# Autodesk Inventor assembly: engine 101 standing model (no movement)
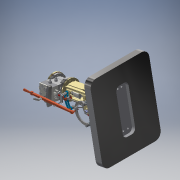
[picture p0: Inventor's stored thumbnail of the model, 180x180]
Saved by Autodesk Inventor 2017 (Build 210142000, 142)
## iProperties
Created: 2018-11-11
Part Number: engine 101 standing model (no movement)
Document SubType Name: Assembly
Designer: User
Author: User
## Documents named in this file (53)
- E:\Sahil's engine\engine 101 standing model (no movement).iam
- E:\Sahil's engine\reverse gear fly wheel.ipt
- E:\Sahil's engine\reverse gear crankshaft outer rod.ipt
- E:\Sahil's engine\reverse gear crankshaft counter weight 2.ipt
- E:\Sahil's engine\reverse gear bearing keeper.ipt
- E:\Sahil's engine\reverse gear connecting rod 1.ipt
- E:\Sahil's engine\reverse gear crankshaft center rod.ipt
- E:\Sahil's engine\reverse gear crank rod 1.ipt
- E:\Sahil's engine\reverse gear crankrod pin 1.ipt
- E:\Sahil's engine\reverse gear cross head 1.ipt
- E:\Sahil's engine\reverse gear pistion rod.ipt
- E:\Sahil's engine\reverse gear piston.ipt
- E:\Sahil's engine\reverse gear  upper base bearing holder 1.ipt
- E:\Sahil's engine\reverse gear lower base bearing holder.ipt
- E:\Sahil's engine\reverse gear lower cylinder ream 1.ipt
- E:\Sahil's engine\reverse gear eccentric 1.ipt
- E:\Sahil's engine\reverse gear base cast 2.ipt
- E:\Sahil's engine\reverse gear stand.ipt
- E:\Sahil's engine\reverse gear lower cylinder cover.ipt
- E:\Sahil's engine\reverse gear cylinder.ipt
- E:\Sahil's engine\reverse gear steam chest.ipt
- E:\Sahil's engine\reverse gear steam chest cover.ipt
- E:\Sahil's engine\reverse gear gear link.ipt
- E:\Sahil's engine\reverse gear link stud.ipt
- C:\Users\User\Documents\engine\Good copy engine Sahil\reverse gear link lever.ipt
- E:\Sahil's engine\reverse gear standard 101.ipt
- E:\Sahil's engine\reverse gear blands.ipt
- C:\Users\User\Documents\engine\Good copy engine Sahil\reverse gear steam chest rod valve.ipt
- E:\Sahil's engine\reverse gear reverse gear.ipt
- E:\Sahil's engine\reverse gear link block.ipt
- E:\Sahil's engine\reverse gear essentric rod 2.ipt
- E:\Sahil's engine\reverse gear trap holders.ipt
- E:\Sahil's engine\reverse gear lower trap.ipt
- E:\Sahil's engine\reverse gear drag link.ipt
- E:\Sahil's engine\reverse gear link rod.ipt
- E:\Sahil's engine\reverse gear lever ring stud.ipt
- E:\Sahil's engine\reverse gear reverse lever ring.ipt
- E:\Sahil's engine\reverse gear cylinder piping connector 2.ipt
- E:\Sahil's engine\reverse gear rever lever.ipt
- C:\Users\User\Documents\Inventor\Content Center Files\R2017\en-US\DIN 84\DIN 84 - M3 x 4.ipt
- C:\Users\User\Documents\Inventor\Content Center Files\R2017\en-US\DIN 84\DIN 84 - M4 x 14.ipt
- C:\Users\User\Documents\Inventor\Content Center Files\R2017\en-US\CNS 4472\CNS 4472 - M 6 x 1.ipt
- C:\Users\User\Documents\Inventor\Content Center Files\R2017\en-US\AS 1421(1)\AS 1421 - M3x5 Cone Point.ipt
- C:\Users\User\Documents\Inventor\Content Center Files\R2017\en-US\AS 1427(03)\AS 1427 - M2.5 x 5(1).ipt
- C:\Users\User\Documents\Inventor\Content Center Files\R2017\en-US\CSN 02 1174  A\CSN 02 1174 - A M3 x 20.ipt
- C:\Users\User\Documents\Inventor\Content Center Files\R2017\en-US\CSN 02 1174  A\CSN 02 1174 - A M3 x 14.ipt
- E:\Sahil's engine\reverse gear up cylinder packing.ipt
- C:\Users\User\Documents\Inventor\Content Center Files\R2017\en-US\AS 1427(03)\AS 1427 - M2 x 10(1).ipt
- E:\Sahil's engine\reverse gear upper cover.ipt
- C:\Users\User\Documents\Inventor\Content Center Files\R2017\en-US\AS 1427(03)\AS 1427 - M2 x 8(1).ipt
- C:\Users\User\Documents\Inventor\Content Center Files\R2017\en-US\AS 1427(03)\AS 1427 - M2 x 6(1).ipt
- C:\Users\User\Documents\Inventor\Content Center Files\R2017\en-US\AS 1427(03)\AS 1427 - M3.5 x 6(1).ipt
- C:\Users\User\Documents\Inventor\Content Center Files\R2017\en-US\AS 1427(03)\AS 1427 - M2 x 20(1).ipt
## Components (109 placed, 52 different names)
1. reverse gear crankshaft outer rod:1 — Insert:2, Insert:21, Rotation:2, Rotation:3
2. reverse gear crankshaft counter weight 2:1 — Insert:2, Rotation:1, Insert:86
3. reverse gear connecting rod 1:2 — Mate:1, Flush:1, Flush:2, Mate:2, Flush:3, Flush:4
4. reverse gear connecting rod 1:3 — Mate:1, Flush:1, Flush:2, Mate:3, Flush:5, Flush:6
5. reverse gear bearing keeper:2 — Mate:2, Flush:3, Flush:4
6. reverse gear crankshaft counter weight 2:2 — Insert:6, Insert:84, Insert:85
7. reverse gear crankshaft outer rod:2 — Insert:6, Insert:12, Insert:14, Insert:15
8. reverse gear crank rod 1:1 — Mate:3, Flush:5, Flush:6, Insert:7, Insert:8, Insert:82, Insert:83
9. reverse gear crankrod pin 1:1 — Insert:7
10. reverse gear cross head 1:1 — Insert:8, Insert:9
11. reverse gear pistion rod:1 — Insert:9, Insert:10, Insert:13
12. reverse gear piston:1 — Insert:10, Insert:30
13. reverse gear  upper base bearing holder 1:1 — Mate:4, Flush:7, Flush:8, Flush:26, Insert:68, Insert:78, Insert:79, Insert:80, Insert:81
14. reverse gear  upper base bearing holder 1:2 — Mate:5, Flush:9, Flush:10, Insert:12, Flush:12, Flush:13, Insert:69, Insert:74, Insert:75, Insert:76, Insert:77, Rotation/Translation:6, Rotation/Translation:7, Rotation/Translation:8, Rotation/Translation:9, Rotation/Translation:10, Rotation/Translation:11, Rotation/Translation:13
15. reverse gear lower base bearing holder:1 — Mate:4, Flush:7, Flush:8, Mate:6, Flush:25, Rotation:1
16. reverse gear lower base bearing holder:2 — Mate:5, Flush:9, Flush:10, Mate:7, Flush:11
17. reverse gear lower cylinder ream 1:1 — Insert:13, Insert:16
18. reverse gear eccentric 1:1 — Insert:14, Insert:31
19. reverse gear eccentric 1:2 — Insert:15, Insert:33
20. reverse gear base cast 2:1 — Mate:6, Mate:7, Flush:11, Flush:12, Flush:13, Mate:8, Flush:14, Flush:15, Flush:20, Flush:21, Flush:22, Flush:25, Flush:26, Insert:41, Insert:43, Rotation:9, Insert:56, Insert:57, Insert:58, Insert:59, Rotation/Translation:14
21. reverse gear stand:1 — Mate:8, Flush:14, Flush:15
22. reverse gear lower cylinder cover:1 — Insert:16
23. reverse gear steam chest:1 — Mate:10, Flush:18, Flush:19, Insert:23, Mate:19, Flush:28, Flush:29, Insert:46
24. reverse gear steam chest cover:1 — Mate:10, Flush:18, Flush:19, Mate:11, Mate:12, Mate:14, Mate:15, Insert:102, Insert:103, Insert:104, Insert:105, Insert:106, Insert:107
25. reverse gear gear link:1 — Mate:11, Mate:12, Mate:14, Mate:15, Rotation:4, Insert:100, Insert:101
26. reverse gear link lever:1 — Rotation:5, Insert:111
27. reverse gear standard 101:1 — Flush:20, Flush:21, Flush:22, Rotation:6, Rotation:7, Insert:50, Insert:51, Insert:52, Insert:53, Insert:54, Insert:55, Rotation:12, Rotation/Translation:1, Rotation/Translation:2, Rotation/Translation:3, Rotation/Translation:4, Rotation/Translation:5, Rotation:15
28. reverse gear fly wheel:1 — Insert:21, Rotation:2, Rotation:3
29. reverse gear blands:1 — Insert:23, Insert:35
30. reverse gear steam chest rod valve:1 — Mate:16, Mate:17, Insert:25, Insert:35
31. reverse gear reverse gear:1 — Insert:26, Insert:28, Rotation:8, Insert:37
32. reverse gear link stud:2 — Insert:25
33. reverse gear link block:1 — Mate:16, Mate:17
34. reverse gear link stud:3 — Insert:26, Insert:36
35. reverse gear link stud:4 — Insert:28, Rotation:8
36. reverse gear cylinder:1 — Insert:30, Mate:19, Flush:28, Flush:29, Rotation:4, Rotation:5, Rotation:6, Rotation:7, Insert:45, Mate:22, Insert:95, Insert:96, Insert:97, Insert:98, Insert:99, Rotation:15
37. reverse gear trap holders:1 — Insert:31, Mate:20, Flush:30, Insert:32, Insert:70, Insert:72
38. reverse gear lower trap:1 — Mate:20, Flush:30
39. reverse gear essentric rod 2:2 — Insert:32, Insert:36
40. reverse gear trap holders:2 — Insert:33, Mate:21, Flush:31, Insert:34, Insert:71, Insert:73
41. reverse gear lower trap:2 — Mate:21, Flush:31
42. reverse gear essentric rod 2:3 — Insert:34
43. reverse gear drag link:1 — Insert:38
44. reverse gear link rod:1 — Insert:37, Insert:38
45. reverse gear reverse lever ring:1 — Insert:42, Rotation:9, Insert:44
46. reverse gear lever ring stud:1 — Insert:41, Insert:42
47. reverse gear lever ring stud:2 — Insert:43
48. reverse gear link stud:6 — Insert:44, Insert:108
49. reverse gear cylinder piping connector 2:1 — Insert:45
50. reverse gear cylinder piping connector 2:2 — Insert:46
51. DIN 84 - replaced by DIN EN ISO 1207 M3 x 4:1 — Insert:50, Rotation:12, Rotation/Translation:1
52. DIN 84 - replaced by DIN EN ISO 1207 M3 x 4:2 — Insert:55, Rotation/Translation:4
53. DIN 84 - replaced by DIN EN ISO 1207 M3 x 4:3 — Insert:54, Rotation/Translation:5
54. DIN 84 - replaced by DIN EN ISO 1207 M3 x 4:4 — Insert:51, Rotation/Translation:2
55. DIN 84 - replaced by DIN EN ISO 1207 M3 x 4:5 — Insert:53
56. DIN 84 - replaced by DIN EN ISO 1207 M3 x 4:6 — Insert:52, Rotation/Translation:3
57. DIN 84 - replaced by DIN EN ISO 1207 M4 x 14:1 — Insert:58, Insert:60
58. DIN 84 - replaced by DIN EN ISO 1207 M4 x 14:2 — Insert:59, Insert:61
59. DIN 84 - replaced by DIN EN ISO 1207 M4 x 14:3 — Insert:56, Insert:62
60. DIN 84 - replaced by DIN EN ISO 1207 M4 x 14:4 — Insert:57, Insert:63
61. CNS 4472 M 6:1 — Insert:60
62. CNS 4472 M 6:2 — Insert:61
63. CNS 4472 M 6:3 — Insert:62
64. CNS 4472 M 6:4 — Insert:63
65. DIN 84 - replaced by DIN EN ISO 1207 M3 x 4:7 — Insert:68
66. DIN 84 - replaced by DIN EN ISO 1207 M3 x 4:8 — Insert:69
67. AS 1421 Cone Point - Metric M3x5 Cone Point:1 — Insert:73
68. AS 1421 Cone Point - Metric M3x5 Cone Point:2 — Insert:71
69. AS 1421 Cone Point - Metric M3x5 Cone Point:3 — Insert:72
70. AS 1421 Cone Point - Metric M3x5 Cone Point:4 — Insert:70
71. AS 1427 - Metric M2.5 x 5:1 — Insert:74, Rotation:14, Rotation/Translation:11, Rotation/Translation:12
72. AS 1427 - Metric M2.5 x 5:2 — Insert:75, Rotation:14, Rotation/Translation:12, Rotation/Translation:13
73. AS 1427 - Metric M2.5 x 5:3 — Insert:76, Rotation/Translation:6, Rotation/Translation:7, Rotation:13
74. AS 1427 - Metric M2.5 x 5:4 — Insert:77, Rotation:13, Rotation/Translation:8, Rotation/Translation:9, Rotation/Translation:10
75. AS 1427 - Metric M2.5 x 5:5 — Insert:78
76. AS 1427 - Metric M2.5 x 5:6 — Insert:80
77. AS 1427 - Metric M2.5 x 5:7 — Insert:79
78. AS 1427 - Metric M2.5 x 5:8 — Insert:81
79. CSN 02 1174 A A M3 x 20:1 — Insert:83
80. CSN 02 1174 A A M3 x 20:2 — Insert:82
81. reverse gear crankshaft center rod:2 — Insert:84
82. CSN 02 1174 A A M3 x 14:1 — Insert:86
83. CSN 02 1174 A A M3 x 14:2 — Insert:85
84. reverse gear up cylinder packing:1 — Mate:22, Mate:23
85. reverse gear upper cover:1 — Mate:23, Insert:87, Insert:88, Insert:89, Insert:90, Insert:91, Insert:92, Insert:93, Insert:94
86. AS 1427 - Metric M2 x 8:1 — Insert:93
87. AS 1427 - Metric M2 x 8:2 — Insert:90
88. AS 1427 - Metric M2 x 8:3 — Insert:88
89. AS 1427 - Metric M2 x 8:4 — Insert:87
90. AS 1427 - Metric M2 x 8:6 — Insert:91
91. AS 1427 - Metric M2 x 8:7 — Insert:92
92. AS 1427 - Metric M2 x 8:8 — Insert:89
93. AS 1427 - Metric M2 x 10:1 — Insert:94
94. AS 1427 - Metric M2 x 6:2 — Insert:97
95. AS 1427 - Metric M2 x 6:4 — Insert:95
96. AS 1427 - Metric M2 x 6:6 — Insert:99
97. AS 1427 - Metric M2 x 6:7 — Insert:98
98. AS 1427 - Metric M2 x 6:8 — Insert:96
99. AS 1427 - Metric M3.5 x 6:1 — Insert:102
100. AS 1427 - Metric M3.5 x 6:2 — Insert:101
101. AS 1427 - Metric M3.5 x 6:3 — Insert:104
102. AS 1427 - Metric M3.5 x 6:4 — Insert:100
103. AS 1427 - Metric M3.5 x 6:5 — Insert:105
104. AS 1427 - Metric M3.5 x 6:6 — Insert:103
105. AS 1427 - Metric M3.5 x 6:7 — Insert:107
106. AS 1427 - Metric M3.5 x 6:8 — Insert:106
107. reverse gear rever lever:1 — Insert:108, Insert:109, Insert:110, Rotation/Translation:14
108. AS 1427 - Metric M2 x 20:1 — Insert:110, Insert:111
109. AS 1427 - Metric M2 x 20:2 — Insert:109
## Relationships (162: Insert 89, Flush 26, Mate 20, RelateRotateTranslate 14, RelateRotation 13)
- Insert:2 (-7 mm): reverse gear crankshaft outer rod:1 ↔ reverse gear crankshaft counter weight 2:1
- Mate:1: reverse gear connecting rod 1:2 ↔ reverse gear connecting rod 1:3
- Flush:1: reverse gear connecting rod 1:2 ↔ reverse gear connecting rod 1:3
- Flush:2: reverse gear connecting rod 1:2 ↔ reverse gear connecting rod 1:3
- Mate:2: reverse gear connecting rod 1:2 ↔ reverse gear bearing keeper:2
- Flush:3: reverse gear connecting rod 1:2 ↔ reverse gear bearing keeper:2
- Flush:4: reverse gear connecting rod 1:2 ↔ reverse gear bearing keeper:2
- Insert:6: reverse gear crankshaft counter weight 2:2 ↔ reverse gear crankshaft outer rod:2
- Mate:3: reverse gear connecting rod 1:3 ↔ reverse gear crank rod 1:1
- Flush:5: reverse gear connecting rod 1:3 ↔ reverse gear crank rod 1:1
- Flush:6: reverse gear connecting rod 1:3 ↔ reverse gear crank rod 1:1
- Insert:7 (-20 mm): reverse gear crank rod 1:1 ↔ reverse gear crankrod pin 1:1
- Insert:8: reverse gear crank rod 1:1 ↔ reverse gear cross head 1:1
- Insert:9 (-7.5 mm): reverse gear cross head 1:1 ↔ reverse gear pistion rod:1
- Insert:10 (7 mm): reverse gear pistion rod:1 ↔ reverse gear piston:1
- Mate:4: reverse gear  upper base bearing holder 1:1 ↔ reverse gear lower base bearing holder:1
- Flush:7 (7 mm): reverse gear  upper base bearing holder 1:1 ↔ reverse gear lower base bearing holder:1
- Flush:8: reverse gear  upper base bearing holder 1:1 ↔ reverse gear lower base bearing holder:1
- Mate:5: reverse gear  upper base bearing holder 1:2 ↔ reverse gear lower base bearing holder:2
- Flush:9 (7 mm): reverse gear  upper base bearing holder 1:2 ↔ reverse gear lower base bearing holder:2
- Flush:10: reverse gear  upper base bearing holder 1:2 ↔ reverse gear lower base bearing holder:2
- Insert:12 (27 mm): reverse gear crankshaft outer rod:2 ↔ reverse gear  upper base bearing holder 1:2
- Insert:13 (-5 mm): reverse gear pistion rod:1 ↔ reverse gear lower cylinder ream 1:1
- Insert:14 (13 mm): reverse gear crankshaft outer rod:2 ↔ reverse gear eccentric 1:1
- Insert:15 (5 mm): reverse gear crankshaft outer rod:2 ↔ reverse gear eccentric 1:2
- Mate:6: reverse gear lower base bearing holder:1 ↔ reverse gear base cast 2:1
- Mate:7: reverse gear lower base bearing holder:2 ↔ reverse gear base cast 2:1
- Flush:11: reverse gear lower base bearing holder:2 ↔ reverse gear base cast 2:1
- Flush:12: reverse gear  upper base bearing holder 1:2 ↔ reverse gear base cast 2:1
- Flush:13 (29 mm): reverse gear  upper base bearing holder 1:2 ↔ reverse gear base cast 2:1
- Mate:8: reverse gear base cast 2:1 ↔ reverse gear stand:1
- Flush:14 (55 mm): reverse gear base cast 2:1 ↔ reverse gear stand:1
- Flush:15 (59 mm): reverse gear base cast 2:1 ↔ reverse gear stand:1
- Insert:16 (1 mm): reverse gear lower cylinder ream 1:1 ↔ reverse gear lower cylinder cover:1
- Mate:10: reverse gear steam chest:1 ↔ reverse gear steam chest cover:1
- Flush:18: reverse gear steam chest:1 ↔ reverse gear steam chest cover:1
- Flush:19: reverse gear steam chest:1 ↔ reverse gear steam chest cover:1
- Mate:11: reverse gear steam chest cover:1 ↔ reverse gear gear link:1
- Mate:12: reverse gear steam chest cover:1 ↔ reverse gear gear link:1
- Flush:20 (12 mm): reverse gear base cast 2:1 ↔ reverse gear standard 101:1
- Flush:21 (0.5 mm): reverse gear base cast 2:1 ↔ reverse gear standard 101:1
- Flush:22 (-3.9 mm): reverse gear base cast 2:1 ↔ reverse gear standard 101:1
- Mate:14: reverse gear steam chest cover:1 ↔ reverse gear gear link:1
- Mate:15: reverse gear steam chest cover:1 ↔ reverse gear gear link:1
- Flush:25: reverse gear lower base bearing holder:1 ↔ reverse gear base cast 2:1
- Flush:26 (29 mm): reverse gear  upper base bearing holder 1:1 ↔ reverse gear base cast 2:1
- Rotation:1 [RelateRotation] (1 ul): reverse gear crankshaft counter weight 2:1 ↔ reverse gear lower base bearing holder:1
- Insert:21 (-8 mm): reverse gear crankshaft outer rod:1 ↔ reverse gear fly wheel:1
- Rotation:2 [RelateRotation] (10.25 ul): reverse gear crankshaft outer rod:1 ↔ reverse gear fly wheel:1
- Rotation:3 [RelateRotation] (10.25 ul): reverse gear crankshaft outer rod:1 ↔ reverse gear fly wheel:1
- Insert:23 (-8 mm): reverse gear steam chest:1 ↔ reverse gear blands:1
- Mate:16: reverse gear steam chest rod valve:1 ↔ reverse gear link block:1
- Mate:17: reverse gear steam chest rod valve:1 ↔ reverse gear link block:1
- Insert:25 (-13 mm): reverse gear steam chest rod valve:1 ↔ reverse gear link stud:2
- Insert:26 (-10 mm): reverse gear reverse gear:1 ↔ reverse gear link stud:3
- Insert:28 (-10 mm): reverse gear reverse gear:1 ↔ reverse gear link stud:4
- Insert:30 (-23 mm): reverse gear piston:1 ↔ reverse gear cylinder:1
- Mate:19: reverse gear steam chest:1 ↔ reverse gear cylinder:1
- Flush:28: reverse gear steam chest:1 ↔ reverse gear cylinder:1
- Flush:29: reverse gear steam chest:1 ↔ reverse gear cylinder:1
- Rotation:4 [RelateRotation] (1 ul): reverse gear gear link:1 ↔ reverse gear cylinder:1
- Rotation:5 [RelateRotation] (1 ul): reverse gear link lever:1 ↔ reverse gear cylinder:1
- Rotation:6 [RelateRotation] (1 ul): reverse gear standard 101:1 ↔ reverse gear cylinder:1
- Rotation:7 [RelateRotation] (1 ul): reverse gear standard 101:1 ↔ reverse gear cylinder:1
- Insert:31 (-1.6 mm): reverse gear eccentric 1:1 ↔ reverse gear trap holders:1
- Mate:20: reverse gear trap holders:1 ↔ reverse gear lower trap:1
- Flush:30: reverse gear trap holders:1 ↔ reverse gear lower trap:1
- Insert:32 (-3 mm): reverse gear trap holders:1 ↔ reverse gear essentric rod 2:2
- Insert:33: reverse gear eccentric 1:2 ↔ reverse gear trap holders:2
- Mate:21: reverse gear trap holders:2 ↔ reverse gear lower trap:2
- Flush:31: reverse gear trap holders:2 ↔ reverse gear lower trap:2
- Insert:34 (-3 mm): reverse gear trap holders:2 ↔ reverse gear essentric rod 2:3
- Insert:35 (-40 mm): reverse gear blands:1 ↔ reverse gear steam chest rod valve:1
- Insert:36 (-6 mm): reverse gear link stud:3 ↔ reverse gear essentric rod 2:2
- Rotation:8 [RelateRotation] (1 ul): reverse gear reverse gear:1 ↔ reverse gear link stud:4
- Insert:37 (4.5 mm): reverse gear reverse gear:1 ↔ reverse gear link rod:1
- Insert:38 (-4 mm): reverse gear drag link:1 ↔ reverse gear link rod:1
- Insert:41: reverse gear base cast 2:1 ↔ reverse gear lever ring stud:1
- Insert:42: reverse gear reverse lever ring:1 ↔ reverse gear lever ring stud:1
- Insert:43: reverse gear base cast 2:1 ↔ reverse gear lever ring stud:2
- Rotation:9 [RelateRotation] (1 ul): reverse gear base cast 2:1 ↔ reverse gear reverse lever ring:1
- Insert:44 (-8 mm): reverse gear reverse lever ring:1 ↔ reverse gear link stud:6
- Insert:45: reverse gear cylinder:1 ↔ reverse gear cylinder piping connector 2:1
- Insert:46 (9 mm): reverse gear steam chest:1 ↔ reverse gear cylinder piping connector 2:2
- Insert:50 (-3.6 mm): reverse gear standard 101:1 ↔ DIN 84 - replaced by DIN EN ISO 1207 M3 x 4:1
- Insert:51 (-3.6 mm): reverse gear standard 101:1 ↔ DIN 84 - replaced by DIN EN ISO 1207 M3 x 4:4
- Insert:52 (-3.6 mm): reverse gear standard 101:1 ↔ DIN 84 - replaced by DIN EN ISO 1207 M3 x 4:6
- Insert:53 (-3.6 mm): reverse gear standard 101:1 ↔ DIN 84 - replaced by DIN EN ISO 1207 M3 x 4:5
- Insert:54 (-3.6 mm): reverse gear standard 101:1 ↔ DIN 84 - replaced by DIN EN ISO 1207 M3 x 4:3
- Insert:55 (-3.6 mm): reverse gear standard 101:1 ↔ DIN 84 - replaced by DIN EN ISO 1207 M3 x 4:2
- Rotation:12 [RelateRotation] (1 ul): reverse gear standard 101:1 ↔ DIN 84 - replaced by DIN EN ISO 1207 M3 x 4:1
- Rotation/Translation:1 [RelateRotateTranslate] (1 mm): reverse gear standard 101:1 ↔ DIN 84 - replaced by DIN EN ISO 1207 M3 x 4:1
- Rotation/Translation:2 [RelateRotateTranslate] (1 mm): reverse gear standard 101:1 ↔ DIN 84 - replaced by DIN EN ISO 1207 M3 x 4:4
- Rotation/Translation:3 [RelateRotateTranslate] (1 mm): reverse gear standard 101:1 ↔ DIN 84 - replaced by DIN EN ISO 1207 M3 x 4:6
- Rotation/Translation:4 [RelateRotateTranslate] (1 mm): reverse gear standard 101:1 ↔ DIN 84 - replaced by DIN EN ISO 1207 M3 x 4:2
- Rotation/Translation:5 [RelateRotateTranslate] (1 mm): reverse gear standard 101:1 ↔ DIN 84 - replaced by DIN EN ISO 1207 M3 x 4:3
- Insert:56 (-12.4 mm): reverse gear base cast 2:1 ↔ DIN 84 - replaced by DIN EN ISO 1207 M4 x 14:3
- Insert:57 (-12.4 mm): reverse gear base cast 2:1 ↔ DIN 84 - replaced by DIN EN ISO 1207 M4 x 14:4
- Insert:58 (-12.8 mm): reverse gear base cast 2:1 ↔ DIN 84 - replaced by DIN EN ISO 1207 M4 x 14:1
- Insert:59 (-12.8 mm): reverse gear base cast 2:1 ↔ DIN 84 - replaced by DIN EN ISO 1207 M4 x 14:2
- Insert:60 (4 mm): DIN 84 - replaced by DIN EN ISO 1207 M4 x 14:1 ↔ CNS 4472 M 6:1
- Insert:61 (-4 mm): DIN 84 - replaced by DIN EN ISO 1207 M4 x 14:2 ↔ CNS 4472 M 6:2
- Insert:62 (-4 mm): DIN 84 - replaced by DIN EN ISO 1207 M4 x 14:3 ↔ CNS 4472 M 6:3
- Insert:63 (-4 mm): DIN 84 - replaced by DIN EN ISO 1207 M4 x 14:4 ↔ CNS 4472 M 6:4
- Insert:68 (-3 mm): reverse gear  upper base bearing holder 1:1 ↔ DIN 84 - replaced by DIN EN ISO 1207 M3 x 4:7
- Insert:69 (-0.8 mm): reverse gear  upper base bearing holder 1:2 ↔ DIN 84 - replaced by DIN EN ISO 1207 M3 x 4:8
- Insert:70 (-3.6 mm): reverse gear trap holders:1 ↔ AS 1421 Cone Point - Metric M3x5 Cone Point:4
- Insert:71: reverse gear trap holders:2 ↔ AS 1421 Cone Point - Metric M3x5 Cone Point:2
- Insert:72: reverse gear trap holders:1 ↔ AS 1421 Cone Point - Metric M3x5 Cone Point:3
- Insert:73 (-4 mm): reverse gear trap holders:2 ↔ AS 1421 Cone Point - Metric M3x5 Cone Point:1
- Insert:74 (-3.9 mm): reverse gear  upper base bearing holder 1:2 ↔ AS 1427 - Metric M2.5 x 5:1
- Insert:75 (-3.9 mm): reverse gear  upper base bearing holder 1:2 ↔ AS 1427 - Metric M2.5 x 5:2
- Insert:76 (-3.9 mm): reverse gear  upper base bearing holder 1:2 ↔ AS 1427 - Metric M2.5 x 5:3
- Insert:77 (-3.9 mm): reverse gear  upper base bearing holder 1:2 ↔ AS 1427 - Metric M2.5 x 5:4
- Insert:78 (-3.9 mm): reverse gear  upper base bearing holder 1:1 ↔ AS 1427 - Metric M2.5 x 5:5
- Insert:79 (-3.9 mm): reverse gear  upper base bearing holder 1:1 ↔ AS 1427 - Metric M2.5 x 5:7
- Insert:80 (-3.9 mm): reverse gear  upper base bearing holder 1:1 ↔ AS 1427 - Metric M2.5 x 5:6
- Insert:81 (-3.9 mm): reverse gear  upper base bearing holder 1:1 ↔ AS 1427 - Metric M2.5 x 5:8
- Insert:82: reverse gear crank rod 1:1 ↔ CSN 02 1174 A A M3 x 20:2
- Insert:83: reverse gear crank rod 1:1 ↔ CSN 02 1174 A A M3 x 20:1
- Insert:84 (-25 mm): reverse gear crankshaft counter weight 2:2 ↔ reverse gear crankshaft center rod:2
- Insert:85 (-1 mm): reverse gear crankshaft counter weight 2:2 ↔ CSN 02 1174 A A M3 x 14:2
- Insert:86 (-1 mm): reverse gear crankshaft counter weight 2:1 ↔ CSN 02 1174 A A M3 x 14:1
- Mate:22: reverse gear cylinder:1 ↔ reverse gear up cylinder packing:1
- Mate:23: reverse gear up cylinder packing:1 ↔ reverse gear upper cover:1
- Insert:87 (-7 mm): reverse gear upper cover:1 ↔ AS 1427 - Metric M2 x 8:4
- Insert:88 (-7 mm): reverse gear upper cover:1 ↔ AS 1427 - Metric M2 x 8:3
- Insert:89 (-7 mm): reverse gear upper cover:1 ↔ AS 1427 - Metric M2 x 8:8
- Insert:90 (-7.5 mm): reverse gear upper cover:1 ↔ AS 1427 - Metric M2 x 8:2
- Insert:91 (-7.5 mm): reverse gear upper cover:1 ↔ AS 1427 - Metric M2 x 8:6
- Insert:92 (-7.5 mm): reverse gear upper cover:1 ↔ AS 1427 - Metric M2 x 8:7
- Insert:93 (-7.5 mm): reverse gear upper cover:1 ↔ AS 1427 - Metric M2 x 8:1
- Insert:94 (-9 mm): reverse gear upper cover:1 ↔ AS 1427 - Metric M2 x 10:1
- Insert:95 (-5 mm): reverse gear cylinder:1 ↔ AS 1427 - Metric M2 x 6:4
- Insert:96 (-5 mm): reverse gear cylinder:1 ↔ AS 1427 - Metric M2 x 6:8
- Insert:97 (-5 mm): reverse gear cylinder:1 ↔ AS 1427 - Metric M2 x 6:2
- Insert:98 (-5 mm): reverse gear cylinder:1 ↔ AS 1427 - Metric M2 x 6:7
- Insert:99 (-5 mm): reverse gear cylinder:1 ↔ AS 1427 - Metric M2 x 6:6
- Insert:100 (-2 mm): reverse gear gear link:1 ↔ AS 1427 - Metric M3.5 x 6:4
- Insert:101: reverse gear gear link:1 ↔ AS 1427 - Metric M3.5 x 6:2
- Insert:102 (-4 mm): reverse gear steam chest cover:1 ↔ AS 1427 - Metric M3.5 x 6:1
- Insert:103 (-4 mm): reverse gear steam chest cover:1 ↔ AS 1427 - Metric M3.5 x 6:6
- Insert:104 (-4 mm): reverse gear steam chest cover:1 ↔ AS 1427 - Metric M3.5 x 6:3
- Insert:105 (-4 mm): reverse gear steam chest cover:1 ↔ AS 1427 - Metric M3.5 x 6:5
- Insert:106 (-4 mm): reverse gear steam chest cover:1 ↔ AS 1427 - Metric M3.5 x 6:8
- Insert:107 (-4 mm): reverse gear steam chest cover:1 ↔ AS 1427 - Metric M3.5 x 6:7
- Insert:108: reverse gear link stud:6 ↔ reverse gear rever lever:1
- Insert:109 (-15 mm): reverse gear rever lever:1 ↔ AS 1427 - Metric M2 x 20:2
- Insert:110 (-14 mm): reverse gear rever lever:1 ↔ AS 1427 - Metric M2 x 20:1
- Insert:111 (-5 mm): reverse gear link lever:1 ↔ AS 1427 - Metric M2 x 20:1
- Rotation/Translation:6 [RelateRotateTranslate] (1 mm): reverse gear  upper base bearing holder 1:2 ↔ AS 1427 - Metric M2.5 x 5:3
- Rotation/Translation:7 [RelateRotateTranslate] (1 mm): reverse gear  upper base bearing holder 1:2 ↔ AS 1427 - Metric M2.5 x 5:3
- Rotation:13 [RelateRotation] (1 ul): AS 1427 - Metric M2.5 x 5:3 ↔ AS 1427 - Metric M2.5 x 5:4
- Rotation/Translation:8 [RelateRotateTranslate] (1 mm): reverse gear  upper base bearing holder 1:2 ↔ AS 1427 - Metric M2.5 x 5:4
- Rotation/Translation:9 [RelateRotateTranslate] (1 mm): reverse gear  upper base bearing holder 1:2 ↔ AS 1427 - Metric M2.5 x 5:4
- Rotation/Translation:10 [RelateRotateTranslate] (13.823 mm): reverse gear  upper base bearing holder 1:2 ↔ AS 1427 - Metric M2.5 x 5:4
- Rotation:14 [RelateRotation] (1 ul): AS 1427 - Metric M2.5 x 5:1 ↔ AS 1427 - Metric M2.5 x 5:2
- Rotation/Translation:11 [RelateRotateTranslate] (1 mm): reverse gear  upper base bearing holder 1:2 ↔ AS 1427 - Metric M2.5 x 5:1
- Rotation/Translation:12 [RelateRotateTranslate] (1 mm): AS 1427 - Metric M2.5 x 5:1 ↔ AS 1427 - Metric M2.5 x 5:2
- Rotation/Translation:13 [RelateRotateTranslate] (13.823 mm): reverse gear  upper base bearing holder 1:2 ↔ AS 1427 - Metric M2.5 x 5:2
- Rotation/Translation:14 [RelateRotateTranslate] (1 mm): reverse gear base cast 2:1 ↔ reverse gear rever lever:1
- Rotation:15 [RelateRotation] (1 ul): reverse gear standard 101:1 ↔ reverse gear cylinder:1
